# Autodesk Inventor assembly: mech_wheel_assembly
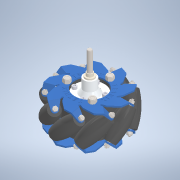
[picture p0: Inventor's stored thumbnail of the model, 180x180]
Saved by Autodesk Inventor 2020 (Build 240168000, 168)
## iProperties
Created: 2019-09-11
Part Number: mech_wheel_assembly
Document SubType Name: Assembly
Designer: tbloo
Author: tbloo
## Documents named in this file (4)
- D:\Documents\GitHub\AO_Robotics\CAD\Projects\Timothy Bloot\mech_wheel_assembly.iam
- D:\Documents\GitHub\AO_Robotics\CAD\Parts Kits\FTC Tetrix KOP Organized (7-24-19)\Wheel\Mechanum Wheel\left_a_mecanum wheel.ipt
- D:\Documents\GitHub\AO_Robotics\CAD\Parts Kits\FTC Tetrix KOP Organized (7-24-19)\Axle Hardware\Tetrix_40225-80mm.ipt
- D:\Documents\GitHub\AO_Robotics\CAD\Parts Kits\FTC Tetrix KOP Organized (7-24-19)\Axle Hardware\AM_6mm_Bushing.ipt
## Components (3 placed, 3 different names)
1. left_a_mecanum wheel:1 — Rigid:1, Rotational:1
2. Tetrix_40225-80mm:1 — Rigid:1
3. AM_6mm_Bushing:1 — Rotational:1
## Relationships (2: WeldJoint 1, RevoluteJoint 1)
- Rigid:1 [WeldJoint]: left_a_mecanum wheel:1 ↔ Tetrix_40225-80mm:1
- Rotational:1 [RevoluteJoint]: left_a_mecanum wheel:1 ↔ AM_6mm_Bushing:1
